# Autodesk Inventor assembly: one side of drive_MIR
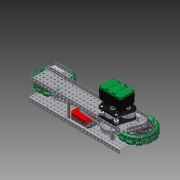
[picture p0: Inventor's stored thumbnail of the model, 180x180]
Saved by Autodesk Inventor 2014 SP1 (Build 180222100, 222)
## iProperties
Created: 2013-10-05
Part Number: one side of drive_MIR
Document SubType Name: Assembly
Designer: RyanHughes
Author: RyanHughes
## Documents named in this file (20)
- C:\Users\Ryan\Desktop\sw\toss up 2ed A bot\drivetrain\one side of drive_MIR.iam
- C:\Users\Ryan\Desktop\sw\lib\Aperture VEX CAD Library\Metal\C Channel\2 x 5.ipt
- C:\Users\Ryan\Desktop\sw\lib\Aperture VEX CAD Library\Bearing Blocks\Bearing Block.ipt
- C:\Users\Ryan\Desktop\sw\lib\Aperture VEX CAD Library\Standoffs\BEAM-2000.ipt
- C:\Users\Ryan\Desktop\sw\lib\Aperture VEX CAD Library\Sprockets\HS Sprockets\18 Tooth HS Sprocket.ipt
- C:\Users\Ryan\Desktop\sw\lib\Aperture VEX CAD Library\Metal\C Channel\5 x 25.ipt
- C:\Users\Ryan\Desktop\sw\toss up 2ed A bot\drivetrain\3 Motor Gearbox.iam
- C:\Users\Ryan\Desktop\sw\lib\Super Sonic Sparks VEX CAD Library\Motors & Sensors\Optical Shaft (Quadrature) Encoder.iam
- C:\Users\Ryan\Desktop\sw\lib\Super Sonic Sparks VEX CAD Library\Gears & Pulleys\12-Tooth Sprocket.ipt
- C:\Users\Ryan\Desktop\sw\lib\Aperture VEX CAD Library\Spacers\SPACER-0500-0125.ipt
- C:\Users\Ryan\Desktop\sw\toss up 2ed A bot\drivetrain\wheel asmby.iam
- C:\Users\Ryan\Desktop\sw\lib\Aperture VEX CAD Library\Spacers\SPACER-0500-0500.ipt
- C:\Users\Ryan\Desktop\sw\toss up 2ed A bot\drivetrain\drive tensioner.iam
- C:\Users\Ryan\Desktop\sw\lib\Aperture VEX CAD Library\Spacers\SPACER-0500-0250.ipt
- C:\Users\Ryan\Desktop\sw\lib\Aperture VEX CAD Library\Hardware\Shaft Collar.ipt
- C:\Users\Ryan\Desktop\sw\lib\Aperture VEX CAD Library\Hardware\8-32\8-32 Nylock_MIR4.ipt
- C:\Users\Ryan\Desktop\sw\toss up 2ed A bot\drivetrain\one side of drive\Design Accelerator\V-Belt transmission1.iam
- C:\Users\Ryan\Desktop\sw\lib\Aperture VEX CAD Library\Sprockets\HS Sprockets\High strength Chain Link.ipt
- C:\Users\Ryan\Desktop\sw\toss up 2ed A bot\drivetrain\one side of drive\Design Accelerator\V-Belt transmission2.iam
- C:\Users\Ryan\Desktop\sw\lib\Aperture VEX CAD Library\Sprockets\Regular Sprockets\CHAIN-LINK.ipt
## Components (198 placed, 18 different names)
1. 2 x 5:1 — Mate:3, Mate:2, Mate:5, Mate:4, Flush:42, Flush:41, Mate:143
2. Bearing Block:1 — Mate:3, Mate:2, Mate:5, Mate:4, Mate:209
3. BEAM-2000:1 — Mate:238, Mate:237, Mate:138
4. Bearing Block:2 — Mate:28, Mate:201, Mate:195, Mate:194, Mate:188
5. 18 Tooth HS Sprocket:1 — Mate:28, Mate:200, Mate:199, Mate:198, Mate:208, Mate:207, Mate:262
6. 2 x 5:2 — Mate:203, Mate:153, Mate:152, Mate:150, Flush:46, Flush:45, Mate:205
7. Bearing Block:3 — Mate:203, Mate:153, Mate:152, Mate:150, Mate:210
8. 2 x 5:3 — Mate:214, Mate:159, Mate:158, Mate:157, Flush:48, Flush:47, Mate:216, Mate:215
9. Bearing Block:4 — Mate:214, Mate:159, Mate:158, Mate:157, Mate:213
10. 5 x 25:1 — Mate:238, Mate:237, Flush:42, Flush:41, Mate:143, Mate:138, Mate:211, Flush:44, Flush:43, Mate:239, Mate:196, Mate:241, Flush:50, Flush:49, Mate:260
11. 5 x 25:2 — Flush:48, Flush:47, Mate:216, Mate:211, Flush:46, Flush:45, Mate:205, Mate:201, Mate:195, Mate:194, Mate:188, Flush:44, Flush:43, Mate:193, Mate:191, Mate:190, Mate:206, Mate:248, Mate:221, Mate:220, Mate:225, Mate:224, Mate:223, Mate:233, Mate:232, Mate:231, Mate:235, Mate:236, Mate:234, Mate:250, Mate:255, Mate:254, Mate:253, Angle:1, Mate:75
12. 3 Motor Gearbox:1 [sub-assembly] — Mate:193, Mate:191, Mate:190, Mate:75
13. Optical Shaft (Quadrature) Encoder:1 [sub-assembly] — Mate:239, Mate:196, Mate:197
14. 12-Tooth Sprocket:1 — Mate:200, Mate:197, Mate:246, Mate:266, Mate:265
15. 12-Tooth Sprocket:2 — Mate:199, Mate:198, Mate:240
16. SPACER-0500-0125:1 — Mate:208, Mate:207, Mate:206
17. wheel asmby:1 [sub-assembly] — Mate:210, Mate:209
18. wheel asmby:2 [sub-assembly] — Mate:215, Mate:213
19. drive tensioner:1 [sub-assembly] — Mate:233, Mate:232, Mate:231
20. drive tensioner:2 [sub-assembly] — Mate:235, Mate:236, Mate:234, Tangent:1
21. SPACER-0500-0500:3 — Mate:241, Mate:240, Mate:243, Mate:242
22. SPACER-0500-0250:1 — Mate:243, Mate:242, Mate:267
23. SPACER-0500-0250:2 — Mate:246, Mate:249
24. SPACER-0500-0250:3 — Mate:250, Mate:249, Mate:252, Mate:251
25. Shaft Collar:1 — Mate:252, Mate:251
26. 8-32 Nylock_MIR4:1 — Mate:255, Mate:254, Mate:253
27. 2 x 5:4 — Flush:50, Flush:49, Mate:260, Mate:261, Mate:257, Mate:256, Mate:259
28. Bearing Block:5 — Mate:261, Mate:257, Mate:256, Mate:259
29. V-Belt transmission:1 [sub-assembly]
30. High strength Chain Link:1 — Tangent:1, Flush:51
31. High strength Chain Link:2
32. High strength Chain Link:3
33. High strength Chain Link:4
34. High strength Chain Link:5
35. High strength Chain Link:6
36. High strength Chain Link:7
37. High strength Chain Link:8
38. High strength Chain Link:9
39. High strength Chain Link:10
40. High strength Chain Link:11
41. High strength Chain Link:12
42. High strength Chain Link:13
43. High strength Chain Link:14
44. High strength Chain Link:15
45. High strength Chain Link:16
46. High strength Chain Link:17
47. High strength Chain Link:18
48. High strength Chain Link:19
49. High strength Chain Link:20
50. High strength Chain Link:21
51. High strength Chain Link:22
52. High strength Chain Link:23
53. High strength Chain Link:24
54. High strength Chain Link:25
55. High strength Chain Link:26
56. High strength Chain Link:27
57. High strength Chain Link:28
58. High strength Chain Link:29
59. High strength Chain Link:30
60. High strength Chain Link:31
61. High strength Chain Link:32
62. High strength Chain Link:33
63. High strength Chain Link:34
64. High strength Chain Link:35
65. High strength Chain Link:36
66. High strength Chain Link:37
67. High strength Chain Link:38
68. High strength Chain Link:39
69. High strength Chain Link:40
70. High strength Chain Link:41
71. High strength Chain Link:42
72. High strength Chain Link:43
73. High strength Chain Link:44
74. High strength Chain Link:45
75. High strength Chain Link:46
76. High strength Chain Link:47
77. High strength Chain Link:48
78. High strength Chain Link:49
79. High strength Chain Link:50
80. High strength Chain Link:51
81. High strength Chain Link:52
82. High strength Chain Link:53
83. High strength Chain Link:54
84. High strength Chain Link:55
85. High strength Chain Link:56
86. High strength Chain Link:57
87. High strength Chain Link:58
88. High strength Chain Link:59
89. High strength Chain Link:60
90. High strength Chain Link:61
91. High strength Chain Link:62
92. High strength Chain Link:63
93. High strength Chain Link:64
94. High strength Chain Link:65
95. High strength Chain Link:66
96. High strength Chain Link:67
97. High strength Chain Link:68
98. High strength Chain Link:69
99. High strength Chain Link:70
100. High strength Chain Link:71
101. High strength Chain Link:72
102. High strength Chain Link:73
103. High strength Chain Link:74 — Flush:52
104. High strength Chain Link:75
105. High strength Chain Link:76
106. High strength Chain Link:77
107. High strength Chain Link:78
108. High strength Chain Link:79
109. High strength Chain Link:80
110. High strength Chain Link:81
111. High strength Chain Link:82
112. High strength Chain Link:83
113. High strength Chain Link:84
114. High strength Chain Link:85
115. V-Belt transmission:2 [sub-assembly]
116. CHAIN-LINK:1 — Mate:267, Mate:266, Mate:265
117. CHAIN-LINK:2
118. CHAIN-LINK:3
119. CHAIN-LINK:4
120. CHAIN-LINK:5
121. CHAIN-LINK:6
122. CHAIN-LINK:7
123. CHAIN-LINK:8
124. CHAIN-LINK:9
125. CHAIN-LINK:10
126. CHAIN-LINK:11
127. CHAIN-LINK:12
128. CHAIN-LINK:13
129. CHAIN-LINK:14
130. CHAIN-LINK:15
131. CHAIN-LINK:16
132. CHAIN-LINK:17
133. CHAIN-LINK:18
134. CHAIN-LINK:19
135. CHAIN-LINK:20
136. CHAIN-LINK:21
137. CHAIN-LINK:22
138. CHAIN-LINK:23
139. CHAIN-LINK:24
140. CHAIN-LINK:25
141. CHAIN-LINK:26
142. CHAIN-LINK:27
143. CHAIN-LINK:28
144. CHAIN-LINK:29
145. CHAIN-LINK:30
146. CHAIN-LINK:31
147. CHAIN-LINK:32
148. CHAIN-LINK:33
149. CHAIN-LINK:34
150. CHAIN-LINK:35
151. CHAIN-LINK:36
152. CHAIN-LINK:37
153. CHAIN-LINK:38
154. CHAIN-LINK:39
155. CHAIN-LINK:40
156. CHAIN-LINK:41
157. CHAIN-LINK:42
158. CHAIN-LINK:43
159. CHAIN-LINK:44
160. CHAIN-LINK:45
161. CHAIN-LINK:46
162. CHAIN-LINK:47
163. CHAIN-LINK:48
164. CHAIN-LINK:49
165. CHAIN-LINK:50
166. CHAIN-LINK:51
167. CHAIN-LINK:52
168. CHAIN-LINK:53
169. CHAIN-LINK:54
170. CHAIN-LINK:55
171. CHAIN-LINK:56
172. CHAIN-LINK:57
173. CHAIN-LINK:58
174. CHAIN-LINK:59
175. CHAIN-LINK:60
176. CHAIN-LINK:61
177. CHAIN-LINK:62
178. CHAIN-LINK:63
179. CHAIN-LINK:64
180. CHAIN-LINK:65
181. CHAIN-LINK:66
182. CHAIN-LINK:67
183. CHAIN-LINK:68
184. CHAIN-LINK:69
185. CHAIN-LINK:70
186. CHAIN-LINK:71
187. CHAIN-LINK:72
188. CHAIN-LINK:73
189. CHAIN-LINK:74
190. CHAIN-LINK:75
191. SPACER-0500-0500:2 — Mate:225, Mate:224, Mate:223
192. SPACER-0500-0500:1 — Mate:248, Mate:221, Mate:220
193. SPACER-0500-0500:4
194. SPACER-0500-0500:5
195. SPACER-0500-0500:6
196. SPACER-0500-0500:7
197. SPACER-0500-0500:8
198. SPACER-0500-0500:9
## Component patterns: (4 elements, first: SPACER-0500-0500:2 + SPACER-0500-0500:1)
## Relationships (88: Mate 72, Flush 14, Tangent 1, Angle 1)
- Mate:3 (2.3114 mm): 2 x 5:1 ↔ Bearing Block:1
- Mate:2: 2 x 5:1 ↔ Bearing Block:1
- Mate:5 (2.3114 mm): 2 x 5:1 ↔ Bearing Block:1
- Mate:4 (2.3114 mm): 2 x 5:1 ↔ Bearing Block:1
- Mate:28: Bearing Block:2 ↔ 18 Tooth HS Sprocket:1
- Mate:203: 2 x 5:2 ↔ Bearing Block:3
- Mate:153 (2.3114 mm): 2 x 5:2 ↔ Bearing Block:3
- Mate:152 (2.3114 mm): 2 x 5:2 ↔ Bearing Block:3
- Mate:150 (2.3114 mm): 2 x 5:2 ↔ Bearing Block:3
- Mate:214: 2 x 5:3 ↔ Bearing Block:4
- Mate:159 (2.3114 mm): 2 x 5:3 ↔ Bearing Block:4
- Mate:158 (2.3114 mm): 2 x 5:3 ↔ Bearing Block:4
- Mate:157 (2.3114 mm): 2 x 5:3 ↔ Bearing Block:4
- Mate:238 (2.3114 mm): BEAM-2000:1 ↔ 5 x 25:1
- Mate:237 (2.3114 mm): BEAM-2000:1 ↔ 5 x 25:1
- Flush:42: 2 x 5:1 ↔ 5 x 25:1
- Flush:41: 2 x 5:1 ↔ 5 x 25:1
- Mate:143: 2 x 5:1 ↔ 5 x 25:1
- Mate:138: BEAM-2000:1 ↔ 5 x 25:1
- Flush:48: 2 x 5:3 ↔ 5 x 25:2
- Flush:47: 2 x 5:3 ↔ 5 x 25:2
- Mate:216: 2 x 5:3 ↔ 5 x 25:2
- Mate:211 (50.8 mm): 5 x 25:1 ↔ 5 x 25:2
- Flush:46: 2 x 5:2 ↔ 5 x 25:2
- Flush:45: 2 x 5:2 ↔ 5 x 25:2
- Mate:205: 2 x 5:2 ↔ 5 x 25:2
- Mate:201: Bearing Block:2 ↔ 5 x 25:2
- Mate:195 (2.3114 mm): Bearing Block:2 ↔ 5 x 25:2
- Mate:194 (2.3114 mm): Bearing Block:2 ↔ 5 x 25:2
- Mate:188 (2.3114 mm): Bearing Block:2 ↔ 5 x 25:2
- Flush:44: 5 x 25:1 ↔ 5 x 25:2
- Flush:43: 5 x 25:1 ↔ 5 x 25:2
- Mate:193 (2.3114 mm): 5 x 25:2 ↔ 3 Motor Gearbox:1
- Mate:191 (2.3114 mm): 5 x 25:2 ↔ 3 Motor Gearbox:1
- Mate:190: 5 x 25:2 ↔ 3 Motor Gearbox:1
- Mate:239 (-0.0614 mm): 5 x 25:1 ↔ Optical Shaft (Quadrature) Encoder:1
- Mate:196: 5 x 25:1 ↔ Optical Shaft (Quadrature) Encoder:1
- Mate:200 [Flush]: 18 Tooth HS Sprocket:1 ↔ 12-Tooth Sprocket:1
- Mate:197: Optical Shaft (Quadrature) Encoder:1 ↔ 12-Tooth Sprocket:1
- Mate:199: 18 Tooth HS Sprocket:1 ↔ 12-Tooth Sprocket:2
- Mate:198 [Flush]: 18 Tooth HS Sprocket:1 ↔ 12-Tooth Sprocket:2
- Mate:208: 18 Tooth HS Sprocket:1 ↔ SPACER-0500-0125:1
- Mate:207: 18 Tooth HS Sprocket:1 ↔ SPACER-0500-0125:1
- Mate:206: 5 x 25:2 ↔ SPACER-0500-0125:1
- Mate:210: Bearing Block:3 ↔ wheel asmby:1
- Mate:209: Bearing Block:1 ↔ wheel asmby:1
- Mate:215: 2 x 5:3 ↔ wheel asmby:2
- Mate:213: Bearing Block:4 ↔ wheel asmby:2
- Mate:248 (2.3114 mm): 5 x 25:2 ↔ SPACER-0500-0500:1
- Mate:221 (2.3114 mm): 5 x 25:2 ↔ SPACER-0500-0500:1
- Mate:220: 5 x 25:2 ↔ SPACER-0500-0500:1
- Mate:225 (2.3114 mm): 5 x 25:2 ↔ SPACER-0500-0500:2
- Mate:224: 5 x 25:2 ↔ SPACER-0500-0500:2
- Mate:223 (2.3114 mm): 5 x 25:2 ↔ SPACER-0500-0500:2
- Mate:233 (2.3114 mm): 5 x 25:2 ↔ drive tensioner:1
- Mate:232 (2.3114 mm): 5 x 25:2 ↔ drive tensioner:1
- Mate:231: 5 x 25:2 ↔ drive tensioner:1
- Mate:235 (2.3114 mm): 5 x 25:2 ↔ drive tensioner:2
- Mate:236 (2.3114 mm): 5 x 25:2 ↔ drive tensioner:2
- Mate:234: 5 x 25:2 ↔ drive tensioner:2
- Mate:241: 5 x 25:1 ↔ SPACER-0500-0500:3
- Mate:240: 12-Tooth Sprocket:2 ↔ SPACER-0500-0500:3
- Mate:243: SPACER-0500-0500:3 ↔ SPACER-0500-0250:1
- Mate:242: SPACER-0500-0500:3 ↔ SPACER-0500-0250:1
- Mate:246: 12-Tooth Sprocket:1 ↔ SPACER-0500-0250:2
- Mate:250: 5 x 25:2 ↔ SPACER-0500-0250:3
- Mate:249: SPACER-0500-0250:2 ↔ SPACER-0500-0250:3
- Mate:252: SPACER-0500-0250:3 ↔ Shaft Collar:1
- Mate:251: SPACER-0500-0250:3 ↔ Shaft Collar:1
- Mate:255: 5 x 25:2 ↔ 8-32 Nylock_MIR4:1
- Mate:254: 5 x 25:2 ↔ 8-32 Nylock_MIR4:1
- Mate:253: 5 x 25:2 ↔ 8-32 Nylock_MIR4:1
- Flush:50: 5 x 25:1 ↔ 2 x 5:4
- Flush:49: 5 x 25:1 ↔ 2 x 5:4
- Mate:260: 5 x 25:1 ↔ 2 x 5:4
- Mate:261 (2.3114 mm): 2 x 5:4 ↔ Bearing Block:5
- Mate:257 (2.3114 mm): 2 x 5:4 ↔ Bearing Block:5
- Mate:256: 2 x 5:4 ↔ Bearing Block:5
- Mate:259 (2.3114 mm): 2 x 5:4 ↔ Bearing Block:5
- Tangent:1 (0.254 mm): drive tensioner:2 ↔ High strength Chain Link:1
- Mate:262 [Flush]: 18 Tooth HS Sprocket:1
- Flush:51 (4.0005 mm): High strength Chain Link:1
- Angle:1 (-13 deg): 5 x 25:2
- Flush:52 [Mate]: High strength Chain Link:74
- Mate:267 (6.35 mm): SPACER-0500-0250:1 ↔ CHAIN-LINK:1
- Mate:266: 12-Tooth Sprocket:1 ↔ CHAIN-LINK:1
- Mate:265: 12-Tooth Sprocket:1 ↔ CHAIN-LINK:1
- Mate:75 (2.3114 mm): 5 x 25:2 ↔ 3 Motor Gearbox:1
## Named parameters: q = 2.3114 mm
